# Autodesk Inventor assembly: corexz
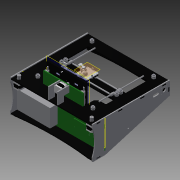
[picture p0: Inventor's stored thumbnail of the model, 180x180]
Saved by Autodesk Inventor 2013 (Build 170138000, 138)
## iProperties
Created: 2014-03-04
Part Number: corexz
Document SubType Name: Assembly
Designer: employee
Author: employee
## Documents named in this file (6)
- C:\Users\employee\Desktop\CoreXZ\corexz.iam
- C:\Users\employee\Desktop\CoreXZ\FRAME.iam
- C:\Users\employee\Desktop\CoreXZ\BED ASSEMBLY.iam
- C:\Users\employee\Desktop\CoreXZ\GANTRY.iam
- C:\Users\employee\Desktop\CoreXZ\EFFECTOR.iam
- C:\Users\employee\Desktop\ConceptFORGE\ConceptFORGE\Wally\INVENTOR\spool.ipt
## Components (5 placed, 5 different names)
1. FRAME:1 [sub-assembly] — Mate:1, Mate:2, Mate:3, Mate:4, Mate:7, Mate:8
2. BED ASSEMBLY:1 [sub-assembly] — Mate:1, Mate:2
3. GANTRY:1 [sub-assembly] — Mate:3, Mate:4, Mate:5, Mate:6
4. EFFECTOR:1 [sub-assembly] — Mate:5, Mate:6
5. spool:1 — Mate:7, Mate:8
## Relationships (8: Mate 8)
- Mate:1: FRAME:1 ↔ BED ASSEMBLY:1
- Mate:2: FRAME:1 ↔ BED ASSEMBLY:1
- Mate:3: FRAME:1 ↔ GANTRY:1
- Mate:4: FRAME:1 ↔ GANTRY:1
- Mate:5: GANTRY:1 ↔ EFFECTOR:1
- Mate:6: GANTRY:1 ↔ EFFECTOR:1
- Mate:7: FRAME:1 ↔ spool:1
- Mate:8: FRAME:1 ↔ spool:1
